# Autodesk Inventor assembly: Assembled Water Sensor Chassi
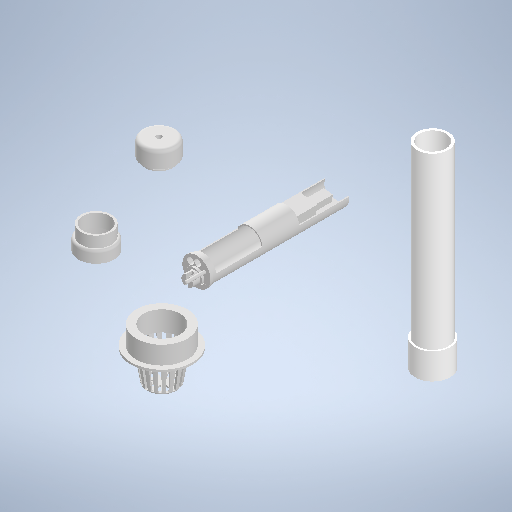
[picture p0: Inventor's stored thumbnail of the model, 512x512]
Saved by Autodesk Inventor 2025 (Build 290162000, 162)
## iProperties
Created: 2024-06-24
Part Number: Assembled Water Sensor Chassi
Document SubType Name: Assembly
Designer: track
Author: track
## Documents named in this file (11)
- C:\Users\track\OneDrive\Documents\In-Situ-Water-Quality-Sensor\System_development\Jocassee\V0.4.7\Bouy_CAD_File\Assembled Water Sensor Chassi.iam
- C:\Users\track\OneDrive\Documents\In-Situ-Water-Quality-Sensor\System_development\Jocassee\V0.4.7\Bouy_CAD_File\Water_Sensor_Cap.ipt
- C:\Users\track\OneDrive\Documents\In-Situ-Water-Quality-Sensor\System_development\Jocassee\V0.4.7\Tray_CAD_File\PCB tray CAD.ipt
- C:\Users\track\OneDrive\Documents\In-Situ-Water-Quality-Sensor\System_development\Jocassee\V0.4.7\Bouy_CAD_File\Water Sensor Shaft (For assembly only).ipt
- C:\Users\track\OneDrive\Documents\Male Adaptor to Water Sensor.ipt
- C:\Users\track\OneDrive\Documents\Water Sensor Grate.ipt
- C:\Users\track\OneDrive\Documents\Arc Water Sensor.ipt
- C:\Users\track\OneDrive\Documents\Light Water Sensor.ipt
- C:\Users\track\OneDrive\Documents\pH Sensor.ipt
- C:\Users\track\OneDrive\Documents\Temp Water Sensor.ipt
- C:\Users\track\OneDrive\Documents\PCB Board.ipt
## Components (10 placed, 10 different names)
1. PCB tray CAD:1 — Flush:2, Mate:2, Flush:3, Mate:3, Mate:4, Mate:5, Rigid:1
2. Water Sensor Shaft (For assembly only):1
3. Water_Sensor_Cap:1
4. Male Adaptor to Water Sensor:1
5. Water Sensor Grate:1
6. Arc Water Sensor:1
7. Light Water Sensor:1 — Flush:3, Rigid:1
8. pH Sensor:1
9. Temp Water Sensor:1 — Flush:2, Mate:2
10. PCB Board:1 — Mate:3, Mate:4, Mate:5
## Relationships (7: Mate 4, Flush 2, WeldJoint 1)
- Flush:2: PCB tray CAD:1 ↔ Temp Water Sensor:1
- Mate:2: PCB tray CAD:1 ↔ Temp Water Sensor:1
- Flush:3: PCB tray CAD:1 ↔ Light Water Sensor:1
- Mate:3: PCB tray CAD:1 ↔ PCB Board:1
- Mate:4: PCB tray CAD:1 ↔ PCB Board:1
- Mate:5: PCB tray CAD:1 ↔ PCB Board:1
- Rigid:1 [WeldJoint]: PCB tray CAD:1 ↔ Light Water Sensor:1
